# Autodesk Inventor assembly: Water Table 4x4
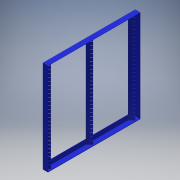
[picture p0: Inventor's stored thumbnail of the model, 180x180]
Saved by Autodesk Inventor 2019 (Build 230136000, 136)
## iProperties
Created: 2017-12-19
Part Number: Water Table 4x4
Document SubType Name: Assembly
Designer: torba
Author: torba
## Documents named in this file (7)
- C:\Users\torba\OneDrive\Documents\Inventor\Plasma 5x10\Water Table 4x4.iam
- C:\Users\torba\OneDrive\Documents\Inventor\Plasma 5x10\3 x 3 angle 45 .25 steel.ipt
- C:\Users\torba\OneDrive\Documents\Inventor\Plasma 5x10\1-16 sheet metal.ipt
- C:\Users\torba\OneDrive\Documents\Inventor\Plasma 5x10\1-16 sheet metal\1-16 sheet metal-48x48.ipt
- C:\Users\torba\OneDrive\Documents\Inventor\Plasma 5x10\3 x 3 angle 45 .25 steel\3 x 3 angle 45 .25 steel-54.ipt
- C:\Users\torba\OneDrive\Documents\Inventor\Plasma 5x10\3 x 3.25 steel\3 x 3 angle 45 .25 steel-54.ipt
- C:\Users\torba\OneDrive\Documents\Inventor\Plasma 5x10\3 x 3.25 steel.ipt
## Components (8 placed, 2 different names)
1. 3 x 3 angle 45 .25 steel-54:1 — Flush:2, Mate:3, Mate:4, Flush:3, Mate:6, Mate:12, Mate:22, Mate:23
2. 3 x 3 angle 45 .25 steel-54:2 — Mate:1, Flush:1, Mate:2, Mate:5, Flush:4, Mate:10, Mate:21
3. 3 x 3 angle 45 .25 steel-54:3 — Mate:1, Flush:1, Mate:2, Flush:2, Mate:3, Mate:4, Mate:17, Mate:18, Mate:19, Mate:20
4. 3 x 3 angle 45 .25 steel-54:4 — Flush:3, Mate:5, Mate:6, Mate:11, Mate:13, Mate:14, Mate:15, Mate:16
5. 1-16 sheet metal-48x48:1 — Flush:4, Mate:10, Mate:11
6. 3 x 3 angle 45 .25 steel-54:1 — Mate:14, Mate:16, Mate:19, Mate:23
7. 3 x 3 angle 45 .25 steel-54:2 — Mate:12, Mate:13, Mate:20, Mate:22
8. 3 x 3 angle 45 .25 steel-54:3 — Mate:15, Mate:17, Mate:18, Mate:21
## Relationships (24: Mate 20, Flush 4)
- Mate:1: 3 x 3 angle 45 .25 steel-54:2 ↔ 3 x 3 angle 45 .25 steel-54:3
- Flush:1: 3 x 3 angle 45 .25 steel-54:2 ↔ 3 x 3 angle 45 .25 steel-54:3
- Mate:2: 3 x 3 angle 45 .25 steel-54:2 ↔ 3 x 3 angle 45 .25 steel-54:3
- Flush:2: 3 x 3 angle 45 .25 steel-54:1 ↔ 3 x 3 angle 45 .25 steel-54:3
- Mate:3: 3 x 3 angle 45 .25 steel-54:1 ↔ 3 x 3 angle 45 .25 steel-54:3
- Mate:4: 3 x 3 angle 45 .25 steel-54:1 ↔ 3 x 3 angle 45 .25 steel-54:3
- Flush:3: 3 x 3 angle 45 .25 steel-54:1 ↔ 3 x 3 angle 45 .25 steel-54:4
- Mate:5: 3 x 3 angle 45 .25 steel-54:2 ↔ 3 x 3 angle 45 .25 steel-54:4
- Mate:6: 3 x 3 angle 45 .25 steel-54:1 ↔ 3 x 3 angle 45 .25 steel-54:4
- Flush:4: 3 x 3 angle 45 .25 steel-54:2 ↔ 1-16 sheet metal-48x48:1
- Mate:10: 3 x 3 angle 45 .25 steel-54:2 ↔ 1-16 sheet metal-48x48:1
- Mate:11: 3 x 3 angle 45 .25 steel-54:4 ↔ 1-16 sheet metal-48x48:1
- Mate:12: 3 x 3 angle 45 .25 steel-54:1 ↔ 3 x 3 angle 45 .25 steel-54:2
- Mate:13: 3 x 3 angle 45 .25 steel-54:4 ↔ 3 x 3 angle 45 .25 steel-54:2
- Mate:14: 3 x 3 angle 45 .25 steel-54:4 ↔ 3 x 3 angle 45 .25 steel-54:1
- Mate:15: 3 x 3 angle 45 .25 steel-54:4 ↔ 3 x 3 angle 45 .25 steel-54:3
- Mate:16: 3 x 3 angle 45 .25 steel-54:4 ↔ 3 x 3 angle 45 .25 steel-54:1
- Mate:17: 3 x 3 angle 45 .25 steel-54:3
- Mate:18: 3 x 3 angle 45 .25 steel-54:3
- Mate:19: 3 x 3 angle 45 .25 steel-54:3 ↔ 3 x 3 angle 45 .25 steel-54:1
- Mate:20: 3 x 3 angle 45 .25 steel-54:3 ↔ 3 x 3 angle 45 .25 steel-54:2
- Mate:21: 3 x 3 angle 45 .25 steel-54:2 ↔ 3 x 3 angle 45 .25 steel-54:3
- Mate:22: 3 x 3 angle 45 .25 steel-54:1 ↔ 3 x 3 angle 45 .25 steel-54:2
- Mate:23 (679.45 mm): 3 x 3 angle 45 .25 steel-54:1
